# Autodesk Inventor assembly: mount
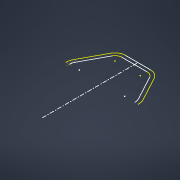
[picture p0: Inventor's stored thumbnail of the model, 180x180]
Saved by Autodesk Inventor 2022 (Build 260153000, 153)
## iProperties
Part Number: mount
Document SubType Name: Assembly
Designer: ancher
Author: ancher
## Documents named in this file (3)
- E:\RC\print_3d\cobrax_mount\mount.iam
- E:\RC\print_3d\cobrax_mount\latch.ipt
- E:\RC\print_3d\cobrax_mount\cap.ipt
## Components (2 placed, 2 different names)
1. latch:1 — Flush:1
2. cap:1 — Flush:1
## Relationships (1: Flush 1)
- Flush:1: latch:1 ↔ cap:1
